# Autodesk Inventor assembly: Air Cylinder 1764
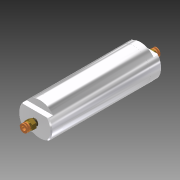
[picture p0: Inventor's stored thumbnail of the model, 180x180]
Saved by Autodesk Inventor 2011 (Build 150239000, 239)
## iProperties
Created: 2010-01-18
Part Number: Air Cylinder 1764
Document SubType Name: Assembly
Designer: cmcfadden
Author: cmcfadden
## Documents named in this file (4)
- R:\CAD Archives\Pneumatics\Air Cylinder 1764\Air Cylinder 1764.iam
- R:\CAD Archives\Pneumatics\Air Cylinder 1764\Air Cylinder Base 1764.ipt
- R:\CAD Archives\Pneumatics\Air Cylinder 1764\Air Cylinder End 1764.ipt
- R:\CAD Archives\Pneumatics\Air Cylinder 1764\Pnewmatic Screw 1764\Pneumatic Screw 1764.iam
## Components (5 placed, 3 different names)
1. Air Cylinder Base 1764:1 — Mate:1, Tangent:1, Mate:2, Tangent:2
2. Air Cylinder End 1764:1 — Mate:1, Tangent:1, Mate:4, Mate:6
3. Air Cylinder End 1764:2 — Mate:2, Tangent:2, Mate:3, Mate:5
4. Pneumatic Screw 1764:1 [sub-assembly] — Mate:3, Mate:5
5. Pneumatic Screw 1764:2 [sub-assembly] — Mate:4, Mate:6
## Relationships (8: Mate 6, Tangent 2)
- Mate:1: Air Cylinder Base 1764:1 ↔ Air Cylinder End 1764:1
- Tangent:1: Air Cylinder Base 1764:1 ↔ Air Cylinder End 1764:1
- Mate:2: Air Cylinder Base 1764:1 ↔ Air Cylinder End 1764:2
- Tangent:2: Air Cylinder Base 1764:1 ↔ Air Cylinder End 1764:2
- Mate:3: Air Cylinder End 1764:2 ↔ Pneumatic Screw 1764:1
- Mate:4: Air Cylinder End 1764:1 ↔ Pneumatic Screw 1764:2
- Mate:5 (3.81 mm): Air Cylinder End 1764:2 ↔ Pneumatic Screw 1764:1
- Mate:6 (3.81 mm): Air Cylinder End 1764:1 ↔ Pneumatic Screw 1764:2
